# Autodesk Inventor assembly: UNLHEP-14-01-A-004_ChuckOnTransportChuck
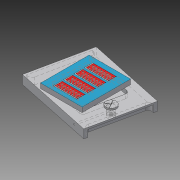
[picture p0: Inventor's stored thumbnail of the model, 180x180]
Saved by Autodesk Inventor 2013 (Build 170138000, 138)
## iProperties
Created: 2014-01-07
Part Number: UNLHEP-14-01-A-004_ChuckOnTransportChuck
Document SubType Name: Assembly
Designer: Frank Meier
Project: UNL Pixel Phase I
Author: Frank Meier
Revision Number: 00
## Documents named in this file (6)
- C:\Users\Frank Meier\Documents\Inventor\Delvotec-Saugplatte\UNLHEP-14-01-A-004_ChuckOnTrspChuck.iam
- C:\Users\Frank Meier\Documents\Inventor\Delvotec-Saugplatte\UNLHEP-14-01-A-003_ChuckW4modules.iam
- C:\Users\Frank Meier\Documents\Inventor\Delvotec-Saugplatte\UNLHEP-14-01-P-007_TransportChuck.ipt
- C:\Users\Frank Meier\Documents\Inventor\Delvotec-Saugplatte\UNLHEP-14-01-P-008_ValveStopper.ipt
- C:\Users\Frank Meier\Documents\Inventor\Content Center Files\R2013\de-DE\DIN 125-1  A\DIN 125 - A 4.3.ipt
- C:\Users\Frank Meier\Documents\Inventor\Content Center Files\R2013\de-DE\DIN 7985 (H)\DIN 7985 (H) - M3x4-H.ipt
## Components (5 placed, 5 different names)
1. UNLHEP-14-01-A-003_ChuckW4modules:1 [sub-assembly] — Fluchtend:1
2. UNLHEP-14-01-P-007_TransportChuck:1 — Fluchtend:1, Einfügen:1
3. UNLHEP-14-01-P-008_ValveStopper:1 — Einfügen:1, Einfügen:2, Passend:1
4. DIN 125-1 A A 4.3:1 — Einfügen:2, Passend:2
5. DIN 7985 (H) M3x4-H:1 — Passend:1, Passend:2
## Relationships (5: Insert 2, Mate 2, Flush 1)
- Fluchtend:1 [Flush]: UNLHEP-14-01-A-003_ChuckW4modules:1 ↔ UNLHEP-14-01-P-007_TransportChuck:1
- Einfügen:1 [Insert]: UNLHEP-14-01-P-007_TransportChuck:1 ↔ UNLHEP-14-01-P-008_ValveStopper:1
- Einfügen:2 [Insert]: UNLHEP-14-01-P-008_ValveStopper:1 ↔ DIN 125-1 A A 4.3:1
- Passend:2 [Mate]: DIN 125-1 A A 4.3:1 ↔ DIN 7985 (H) M3x4-H:1
- Passend:1 [Mate]: UNLHEP-14-01-P-008_ValveStopper:1 ↔ DIN 7985 (H) M3x4-H:1
